# Autodesk Inventor assembly: SC-6-F
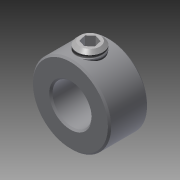
[picture p0: Inventor's stored thumbnail of the model, 180x180]
Saved by Autodesk Inventor 2013 (Build 170138000, 138)
## iProperties
Category: Miscellaneous
Company: Autodesk Inc.
Created: 2012-12-03
Part Number: SC-6-F
Document SubType Name: Assembly
Designer: Autodesk Inc.
Catalog Web Link: http://www.ruland.com/ps_collars_shaft_sc.asp
Description: 3/8" ID 3/4" OD shaft collar
Vendor: Ruland Manufacturing
Author: Autodesk Inc.
## Documents named in this file (3)
- C:\Data Folder\FIRST 2013\FIRST KOP\Parts\Miscellaneous\MISC_ShaftCollar_SC-6-F.iam
- C:\Data Folder\FIRST 2013\FIRST KOP\Parts\Miscellaneous\MISC_ShaftCollar_SC-6-F.ipt
- C:\Data Folder\FIRST 2013\FIRST KOP\Parts\Miscellaneous\ANSI B18.3 - 1_4-20 UNC - 0.25(24).ipt
## Components (2 placed, 2 different names)
1. MISC_ShaftCollar_SC-6-F:1 — Mate:1
2. Hexagon Socket Set Screw - Flat Point - Inch 1/4-20 UNC x 0.25:1 — Mate:1
## Relationships (1: Mate 1)
- Mate:1: MISC_ShaftCollar_SC-6-F:1 ↔ Hexagon Socket Set Screw - Flat Point - Inch 1/4-20 UNC x 0.25:1
